# Autodesk Inventor assembly: MOGO Funnel
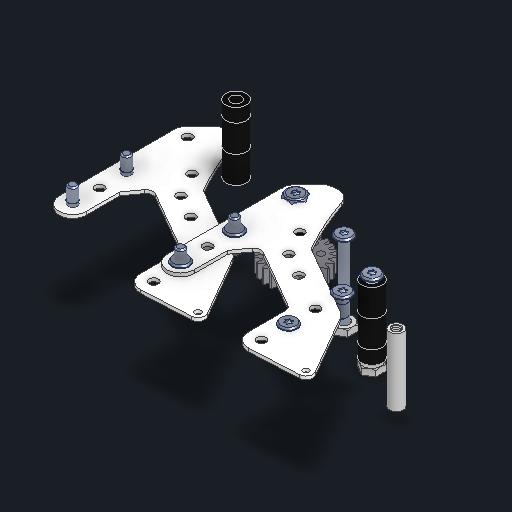
[picture p0: Inventor's stored thumbnail of the model, 512x512]
Saved by Autodesk Inventor 2025.1 (Build 291241000, 241)
## iProperties
Created: 2024-11-13
Part Number: MOGO Funnel
Document SubType Name: Assembly
Designer: avere
Author: avere
## Documents named in this file (17)
- C:\Users\avere\VEX\High Stakes\CAD\V3\Chassis\Drivebay Right\MOGO Funnel.iam
- C:\Users\avere\VEX\High Stakes\CAD\V3\Chassis\Drivebay Left\Custom Parts\MOGO Funnel Gusset.ipt
- C:\Users\avere\VEX\High Stakes\CAD\V3\Chassis\Drivebay Right\Half Cut HS 24T Gear, No Insert.ipt
- C:\Users\avere\VEX\High Stakes\CAD\V3\Chassis\Drivebay Right\Nut Keps.ipt
- C:\Users\avere\VEX\High Stakes\CAD\ROBOPROS-CAD-Inventor\Motion\Spacers\Spacer Nylon .375 OD\NSpacer .375 OD x .250.ipt
- C:\Users\avere\VEX\High Stakes\CAD\ROBOPROS-CAD-Inventor\Motion\Spacers\Spacer Nylon .375 OD.ipt
- C:\Users\avere\VEX\High Stakes\CAD\ROBOPROS-CAD-Inventor\Motion\Spacers\Washer Teflon\TWasher .375 OD x .04000.ipt
- C:\Users\avere\VEX\High Stakes\CAD\ROBOPROS-CAD-Inventor\Motion\Spacers\Washer Teflon.ipt
- C:\Users\avere\VEX\High Stakes\CAD\ROBOPROS-CAD-Inventor\Motion\Spacers\Washer Steel\SWasher .375 OD x .015625.ipt
- C:\Users\avere\VEX\High Stakes\CAD\ROBOPROS-CAD-Inventor\Motion\Spacers\Washer Steel.ipt
- C:\Users\avere\VEX\High Stakes\CAD\ROBOPROS-CAD-Inventor\Motion\Spacers\Spacer Nylon .375 OD\NSpacer .375 OD x .500.ipt
- C:\Users\avere\VEX\High Stakes\CAD\V3\Chassis\Drivebay Right\Nut Nylon Thread-Forming.ipt
- C:\Users\avere\VEX\High Stakes\CAD\ROBOPROS-CAD-Inventor\Structure\Hardware\Screw Steel - Star\SScrew Star Smooth 1.500.ipt
- C:\Users\avere\VEX\High Stakes\CAD\ROBOPROS-CAD-Inventor\Structure\Hardware\Screw Steel - Star.ipt
- C:\Users\avere\VEX\High Stakes\CAD\ROBOPROS-CAD-Inventor\Structure\Nylon Standoff Rounded\Nylon Standoff 1.250.ipt
- C:\Users\avere\VEX\High Stakes\CAD\ROBOPROS-CAD-Inventor\Structure\Hardware\Screw Shoulder Robosource\SScrew Shoulder Smooth .375 x .12.ipt
- C:\Users\avere\VEX\High Stakes\CAD\ROBOPROS-CAD-Inventor\Structure\Hardware\Screw Shoulder Robosource.ipt
## Components (29 placed, 11 different names)
1. MOGO Funnel Gusset:1 — Mate:1, Insert:18, Insert:24
2. MOGO Funnel Gusset:2 — Mate:1, Insert:19, Insert:21, Insert:23
3. Half Cut HS 24T Gear, No Insert:1
4. Nut Keps:1
5. TWasher .375 OD x .04000:1
6. TWasher .375 OD x .04000:2 — Insert:8
7. SWasher .375 OD x .015625:1 — Insert:9
8. NSpacer .375 OD x .500:2 — Insert:8, Insert:9
9. Nut Nylon Thread-Forming:1
10. Nut Nylon Thread-Forming:2
11. Nut Nylon Thread-Forming:3
12. NSpacer .375 OD x .500:4 — Insert:13
13. NSpacer .375 OD x .500:5 — Insert:13, Insert:14
14. NSpacer .375 OD x .250:6 — Insert:14
15. NSpacer .375 OD x .500:7 — Insert:18
16. NSpacer .375 OD x .500:8
17. NSpacer .375 OD x .250:9
18. SScrew Star Smooth 1.500:1
19. SScrew Star Smooth 1.500:2 — Insert:19
20. SScrew Star Smooth 1.500:3 — Insert:21
21. Nylon Standoff 1.250:1
22. SScrew Shoulder Smooth .375 x .12:1 — Insert:23
23. SScrew Shoulder Smooth .375 x .12:2
24. SScrew Shoulder Smooth .375 x .12:3
25. SScrew Shoulder Smooth .375 x .12:4
26. SScrew Shoulder Smooth .375 x .12:5 — Insert:24
27. SScrew Shoulder Smooth .375 x .12:6
28. SScrew Shoulder Smooth .375 x .12:7
29. SScrew Shoulder Smooth .375 x .12:8
## Component patterns: (4 elements, first: SScrew Shoulder Smooth .375 x .12:1), (4 elements, first: SScrew Shoulder Smooth .375 x .12:5)
## Relationships (15: Insert 14, Mate 1)
- Mate:1: MOGO Funnel Gusset:1 ↔ MOGO Funnel Gusset:2
- [Insert]: TWasher .375 OD x .04000:1 ↔ SWasher .375 OD x .015625:1
- [Insert]: Half Cut HS 24T Gear, No Insert:1 ↔ TWasher .375 OD x .04000:1
- [Insert]: Nut Keps:1 ↔ TWasher .375 OD x .04000:2
- Insert:8: TWasher .375 OD x .04000:2 ↔ NSpacer .375 OD x .500:2
- Insert:9: SWasher .375 OD x .015625:1 ↔ NSpacer .375 OD x .500:2
- Insert:13: NSpacer .375 OD x .500:4 ↔ NSpacer .375 OD x .500:5
- Insert:14: NSpacer .375 OD x .500:5 ↔ NSpacer .375 OD x .250:6
- [Insert]: NSpacer .375 OD x .500:7 ↔ NSpacer .375 OD x .500:8
- [Insert]: NSpacer .375 OD x .500:8 ↔ NSpacer .375 OD x .250:9
- Insert:18: MOGO Funnel Gusset:1 ↔ NSpacer .375 OD x .500:7
- Insert:19: MOGO Funnel Gusset:2 ↔ SScrew Star Smooth 1.500:2
- Insert:21: MOGO Funnel Gusset:2 ↔ SScrew Star Smooth 1.500:3
- Insert:23: MOGO Funnel Gusset:2 ↔ SScrew Shoulder Smooth .375 x .12:1
- Insert:24: MOGO Funnel Gusset:1 ↔ SScrew Shoulder Smooth .375 x .12:5
## Named parameters: d17_d13 = 0 mm, d18_d15 = 0 mm
